# Autodesk Inventor assembly: QR_Ramenschraube_unten_M6x60
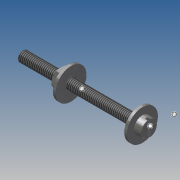
[picture p0: Inventor's stored thumbnail of the model, 180x180]
Saved by Autodesk Inventor 2015 SP1 (Build 190203100, 203)
## iProperties
Created: 2015-03-05
Part Number: QR_Ramenschraube_unten_M6x60
Document SubType Name: Assembly
Designer: Marc
Author: Marc
## Documents named in this file (4)
- E:\Modellflieger\3D Drucker\Eigene Teile\Eigene Schrauben\QR_Ramenschraube_unten_M6x60.iam
- C:\Users\Marc\Documents\Inventor\Content Center Files\R2015\de-DE\DIN 9021\DIN 9021 - 6,4.ipt
- C:\Users\Marc\Documents\Inventor\Content Center Files\R2015\de-DE\DIN 934\DIN 934 - M6 x 1.ipt
- E:\Modellflieger\3D Drucker\Eigene Teile\Eigene Schrauben\DIN 84 - M6 x 70.ipt
## Components (4 placed, 3 different names)
1. DIN 84 - M6 x 70:1
2. DIN 9021 6,4:1
3. DIN 9021 6,4:2
4. DIN 934 - ersetzt durch DIN EN 24032/28673/28674 M6:1
## Relationships (4: Insert 2, Mate 2)
- [Insert]: DIN 84 - M6 x 70:1 ↔ DIN 9021 6,4:1
- [Insert] (-28.4 mm): DIN 84 - M6 x 70:1 ↔ DIN 9021 6,4:2
- [Mate]: DIN 84 - M6 x 70:1 ↔ DIN 934 - ersetzt durch DIN EN 24032/28673/28674 M6:1
- [Mate]: DIN 9021 6,4:2 ↔ DIN 934 - ersetzt durch DIN EN 24032/28673/28674 M6:1
